# Autodesk Inventor assembly: S4x3
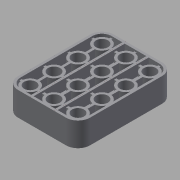
[picture p0: Inventor's stored thumbnail of the model, 180x180]
Saved by Autodesk Inventor 2019.3 (Build 233278000, 278)
## iProperties
Created: 2019-01-31
Part Number: S4x3
Document SubType Name: Assembly
Designer: Varga Daniel
Author: Varga Daniel
## Documents named in this file (6)
- C:\!_Dani\!_cloud\OneDrive\!_munka\Revolution\RevvyDemoKit\Structural parts\Beams\Straight Beams\S3+x3+\S4x3.iam
- C:\!_Dani\!_cloud\OneDrive\!_munka\Revolution\RevvyDemoKit\Structural parts\Beams\beam_side_part.ipt
- C:\!_Dani\!_cloud\OneDrive\!_munka\Revolution\RevvyDemoKit\Structural parts\Beams\beam_inner_part.ipt
- C:\!_Dani\!_cloud\OneDrive\!_munka\Revolution\RevvyDemoKit\Structural parts\Beams\beam_corner_part.ipt
- C:\!_Dani\!_cloud\OneDrive\!_munka\Revolution\RevvyDemoKit\Structural parts\Beams\beam_top_bot_part.ipt
- C:\!_Dani\!_cloud\OneDrive\!_munka\Revolution\RevvyDemoKit\Structural parts\Beams\Straight Beams\S3+x3+.iam
## Components (12 placed, 4 different names)
1. beam_corner_part:1 — Flush:1, Flush:2, Mate:1, Flush:3, Flush:4, Mate:2, Flush:5, Flush:6, Flush:11, Flush:12, Mate:5, Mate:8
2. beam_corner_part:2 — Mate:1, Flush:3, Flush:4
3. beam_corner_part:3 — Flush:11, Flush:12, Mate:5, Flush:13, Flush:14, Mate:6, Flush:15, Flush:16, Mate:7
4. beam_corner_part:4 — Flush:13, Flush:14, Mate:6
5. beam_top_bot_part:1 — Flush:1, Flush:2, Mate:2
6. beam_top_bot_part:3 — Flush:15, Flush:16, Mate:7
7. beam_side_part:2 — Flush:7, Flush:8, Mate:3
8. beam_side_part:1 — Flush:5, Flush:6, Flush:7, Flush:8, Mate:3, Flush:9, Flush:10, Mate:4, Mate:8
9. beam_side_part:3
10. beam_side_part:4
11. beam_inner_part:1 — Flush:9, Flush:10, Mate:4
12. beam_inner_part:3
## Component patterns: (1 elements, first: beam_top_bot_part:1), (1 elements, first: beam_top_bot_part:3), (2 elements, first: beam_side_part:2 + beam_side_part:1), (1 elements, first: beam_inner_part:1), Component Pattern 6:2 (1 elements)
## Relationships (24: Flush 16, Mate 8)
- Flush:1: beam_corner_part:1 ↔ beam_top_bot_part:1
- Flush:2: beam_corner_part:1 ↔ beam_top_bot_part:1
- Mate:1 (10 mm): beam_corner_part:1 ↔ beam_corner_part:2
- Flush:3: beam_corner_part:1 ↔ beam_corner_part:2
- Flush:4: beam_corner_part:1 ↔ beam_corner_part:2
- Mate:2: beam_corner_part:1 ↔ beam_top_bot_part:1
- Flush:5: beam_corner_part:1 ↔ beam_side_part:1
- Flush:6: beam_corner_part:1 ↔ beam_side_part:1
- Flush:7: beam_side_part:2 ↔ beam_side_part:1
- Flush:8: beam_side_part:2 ↔ beam_side_part:1
- Mate:3 (10 mm): beam_side_part:2 ↔ beam_side_part:1
- Flush:9: beam_side_part:1 ↔ beam_inner_part:1
- Flush:10: beam_side_part:1 ↔ beam_inner_part:1
- Mate:4: beam_side_part:1 ↔ beam_inner_part:1
- Flush:11: beam_corner_part:1 ↔ beam_corner_part:3
- Flush:12: beam_corner_part:1 ↔ beam_corner_part:3
- Mate:5 (20 mm): beam_corner_part:1 ↔ beam_corner_part:3
- Flush:13: beam_corner_part:3 ↔ beam_corner_part:4
- Flush:14: beam_corner_part:3 ↔ beam_corner_part:4
- Mate:6 (10 mm): beam_corner_part:3 ↔ beam_corner_part:4
- Flush:15: beam_corner_part:3 ↔ beam_top_bot_part:3
- Flush:16: beam_corner_part:3 ↔ beam_top_bot_part:3
- Mate:7: beam_corner_part:3 ↔ beam_top_bot_part:3
- Mate:8: beam_corner_part:1 ↔ beam_side_part:1
